# Autodesk Inventor assembly: V-Wheel Kit
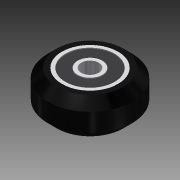
[picture p0: Inventor's stored thumbnail of the model, 180x180]
Saved by Autodesk Inventor 2014 SP1 (Build 180222100, 222)
## iProperties
Created: 2016-04-10
Part Number: V-Wheel Kit
Document SubType Name: Assembly
Designer: Ben
Author: Ben
## Documents named in this file (4)
- C:\Users\Ben\Documents\Autodesk\Projects\Me\3D printer\stp hardware\V-Wheel Kit\V-Wheel Kit.iam
- C:\Users\Ben\Documents\Autodesk\Projects\Me\3D printer\carriages\Solid V-Wheel.ipt
- C:\Users\Ben\Documents\Autodesk\Projects\Me\3D printer\carriages\Ball Bearing 625 2RS 5x16x5.ipt
- C:\Users\Ben\Documents\Autodesk\Projects\Me\3D printer\carriages\1mm 5mm shim.ipt
## Components (4 placed, 3 different names)
1. Solid V-Wheel:1 — Mate:1, Mate:2, Flush:1
2. Ball Bearing 625 2RS 5x16x5:1 — Mate:1, Mate:3, Mate:4, Mate:5
3. Ball Bearing 625 2RS 5x16x5:2 — Mate:2, Mate:3, Flush:1
4. 1mm 5mm shim:1 — Mate:4, Mate:5
## Relationships (6: Mate 5, Flush 1)
- Mate:1: Solid V-Wheel:1 ↔ Ball Bearing 625 2RS 5x16x5:1
- Mate:2: Solid V-Wheel:1 ↔ Ball Bearing 625 2RS 5x16x5:2
- Mate:3: Ball Bearing 625 2RS 5x16x5:1 ↔ Ball Bearing 625 2RS 5x16x5:2
- Flush:1: Solid V-Wheel:1 ↔ Ball Bearing 625 2RS 5x16x5:2
- Mate:4: Ball Bearing 625 2RS 5x16x5:1 ↔ 1mm 5mm shim:1
- Mate:5: Ball Bearing 625 2RS 5x16x5:1 ↔ 1mm 5mm shim:1
